# Autodesk Inventor assembly: Assembly
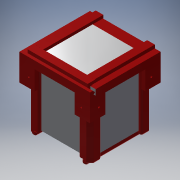
[picture p0: Inventor's stored thumbnail of the model, 180x180]
Saved by Autodesk Inventor 2018 (Build 220112000, 112)
## iProperties
Created: 2019-10-03
Part Number: Assembly
Document SubType Name: Assembly
Designer: Ivan
Author: Ivan
## Documents named in this file (6)
- C:\Users\Ivan\Documents\GitHub\Sensor-de-Vibraciones\Faraday\Assembly.iam
- C:\Users\Ivan\Documents\GitHub\Sensor-de-Vibraciones\Faraday\Bottom.ipt
- C:\Users\Ivan\Documents\GitHub\Sensor-de-Vibraciones\Faraday\TopBox.ipt
- C:\Users\Ivan\Documents\GitHub\Sensor-de-Vibraciones\Faraday\Flat52.ipt
- C:\Users\Ivan\Documents\GitHub\Sensor-de-Vibraciones\Faraday\Flat60.ipt
- C:\Users\Ivan\Documents\GitHub\Sensor-de-Vibraciones\Faraday\SlidingLock.ipt
## Components (10 placed, 5 different names)
1. Bottom:1 — Insert:1, Insert:2, Flush:1, Mate:5, Mate:9, Mate:12, Mate:15, Mate:16, Mate:17, Mate:18, Mate:19, Mate:20, Mate:21, Mate:22, Mate:23, Mate:25
2. TopBox:1 — Insert:1, Insert:2, Mate:1, Mate:2, Mate:3, Mate:4, Mate:6, Mate:7, Mate:8, Mate:10, Mate:11
3. Flat52:1 — Mate:1, Mate:2, Mate:3
4. Flat60:1 — Mate:4, Mate:5, Mate:6
5. Flat60:2 — Mate:7, Mate:8, Mate:9
6. Flat60:3 — Mate:10, Mate:11, Mate:12
7. SlidingLock:1 — Mate:18, Mate:19, Mate:20, Mate:27
8. SlidingLock:2 — Mate:15, Mate:16, Mate:17
9. SlidingLock:3 — Mate:21, Mate:22, Mate:23, Mate:26
10. Flat52:2 — Mate:25, Mate:26, Mate:27
## Relationships (27: Mate 24, Insert 2, Flush 1)
- Insert:1: Bottom:1 ↔ TopBox:1
- Insert:2: Bottom:1 ↔ TopBox:1
- Flush:1: Bottom:1
- Mate:1: TopBox:1 ↔ Flat52:1
- Mate:2: TopBox:1 ↔ Flat52:1
- Mate:3: TopBox:1 ↔ Flat52:1
- Mate:4: TopBox:1 ↔ Flat60:1
- Mate:5: Bottom:1 ↔ Flat60:1
- Mate:6: TopBox:1 ↔ Flat60:1
- Mate:7: TopBox:1 ↔ Flat60:2
- Mate:8: TopBox:1 ↔ Flat60:2
- Mate:9: Bottom:1 ↔ Flat60:2
- Mate:10: TopBox:1 ↔ Flat60:3
- Mate:11: TopBox:1 ↔ Flat60:3
- Mate:12: Bottom:1 ↔ Flat60:3
- Mate:15: Bottom:1 ↔ SlidingLock:2
- Mate:16: Bottom:1 ↔ SlidingLock:2
- Mate:17: Bottom:1 ↔ SlidingLock:2
- Mate:18: Bottom:1 ↔ SlidingLock:1
- Mate:19: Bottom:1 ↔ SlidingLock:1
- Mate:20: Bottom:1 ↔ SlidingLock:1
- Mate:21: Bottom:1 ↔ SlidingLock:3
- Mate:22: Bottom:1 ↔ SlidingLock:3
- Mate:23: Bottom:1 ↔ SlidingLock:3
- Mate:25: Bottom:1 ↔ Flat52:2
- Mate:26: SlidingLock:3 ↔ Flat52:2
- Mate:27: SlidingLock:1 ↔ Flat52:2
